# Autodesk Inventor assembly: Escenario2
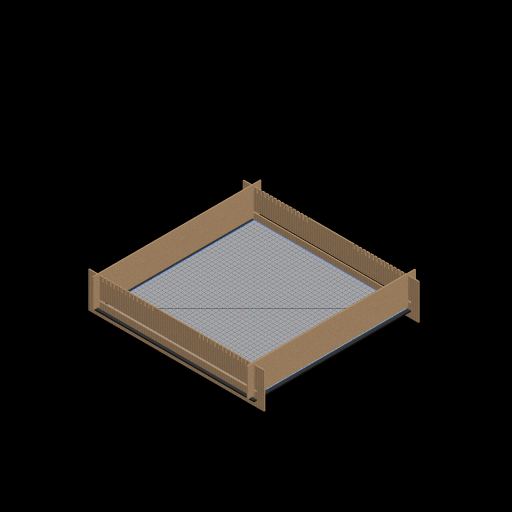
[picture p0: Inventor's stored thumbnail of the model, 512x512]
Saved by Autodesk Inventor 2024.2 (Build 282272000, 272)
## iProperties
Created: 2024-11-02
Part Number: Escenario2
Document SubType Name: Assembly
Designer: jrcer
Author: jrcer
## Documents named in this file (5)
- C:\Users\jrcer\Universidad\S10_2024\TDG\Tesis\Modelos\Escenario2.iam
- C:\Users\jrcer\Universidad\S10_2024\TDG\Tesis\Modelos\C41x41.ipt
- C:\Users\jrcer\Universidad\S10_2024\TDG\Tesis\Modelos\Pared.ipt
- C:\Users\jrcer\Universidad\S10_2024\TDG\Tesis\Modelos\Pared40.ipt
- C:\Users\jrcer\Universidad\S10_2024\TDG\Tesis\Modelos\Cuadricula40X40.ipt
## Components (6 placed, 4 different names)
1. C41x41:1 — Mate:1, Mate:2, Mate:3, Mate:4, Mate:5, Mate:6, Mate:13, Flush:1, Flush:2
2. Pared:1 — Mate:1, Mate:2, Mate:3, Mate:10
3. Pared:2 — Mate:4, Mate:5, Mate:6, Mate:7, Mate:8, Mate:9, Mate:11, Mate:12
4. Pared40:1 — Mate:7, Mate:8, Mate:9
5. Pared40:2 — Mate:10, Mate:11, Mate:12
6. Cuadricula40X40:1 — Mate:13, Flush:1, Flush:2
## Relationships (15: Mate 13, Flush 2)
- Mate:1 (-10 mm): C41x41:1 ↔ Pared:1
- Mate:2: C41x41:1 ↔ Pared:1
- Mate:3: C41x41:1 ↔ Pared:1
- Mate:4 (-10 mm): C41x41:1 ↔ Pared:2
- Mate:5: C41x41:1 ↔ Pared:2
- Mate:6: C41x41:1 ↔ Pared:2
- Mate:7: Pared:2 ↔ Pared40:1
- Mate:8: Pared:2 ↔ Pared40:1
- Mate:9: Pared:2 ↔ Pared40:1
- Mate:10: Pared:1 ↔ Pared40:2
- Mate:11: Pared:2 ↔ Pared40:2
- Mate:12: Pared:2 ↔ Pared40:2
- Mate:13: C41x41:1 ↔ Cuadricula40X40:1
- Flush:1 (10 mm): C41x41:1 ↔ Cuadricula40X40:1
- Flush:2 (10 mm): C41x41:1 ↔ Cuadricula40X40:1
